# Autodesk Inventor assembly: Fuel Assembly
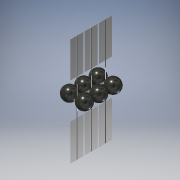
[picture p0: Inventor's stored thumbnail of the model, 180x180]
Saved by Autodesk Inventor 2017.2 (Build 212233000, 233)
## iProperties
Created: 2017-03-31
Part Number: Fuel Assembly
Document SubType Name: Assembly
Designer: haden
Author: haden
## Documents named in this file (5)
- C:\Users\haden\Desktop\Asteroid-Mining-Project\CAD model\Storage Module\Fuel Assembly.iam
- C:\Users\haden\Desktop\Asteroid-Mining-Project\CAD model\Storage Module\Fuel Distributor.ipt
- C:\Users\haden\Desktop\Asteroid-Mining-Project\CAD model\Storage Module\Tube connection.ipt
- C:\Users\haden\Desktop\Asteroid-Mining-Project\CAD model\Storage Module\Tank.ipt
- C:\Users\haden\Desktop\Asteroid-Mining-Project\CAD model\Solar Module\Solar Array.iam
## Components (19 placed, 4 different names)
1. Fuel Distributor:1 — Mate:1, Mate:2, Mate:3, Mate:4, Mate:5, Mate:6, Mate:7, Mate:8, Insert:7, Insert:8, Insert:9, Insert:10, Insert:11, Insert:12
2. Tube connection:1 — Mate:3, Flush:1, Mate:7, Insert:4
3. Tube connection:2 — Mate:2, Flush:1, Flush:2, Insert:5
4. Tube connection:3 — Mate:1, Flush:2, Insert:6
5. Tube connection:4 — Mate:4, Flush:3, Insert:3
6. Tube connection:5 — Mate:5, Flush:3, Flush:4, Insert:2
7. Tube connection:6 — Mate:6, Flush:4, Mate:8, Insert:1
8. Tank:1 — Insert:3
9. Tank:2 — Insert:2
10. Tank:3 — Insert:1
11. Tank:4 — Insert:4
12. Tank:5 — Insert:5
13. Tank:6 — Insert:6
14. Solar Array:1 [sub-assembly] — Insert:7, Angle:1, Angle:2, Angle:3
15. Solar Array:2 [sub-assembly] — Insert:8, Angle:1, Angle:2, Angle:3, Angle:4
16. Solar Array:3 [sub-assembly] — Insert:9, Angle:4, Angle:5
17. Solar Array:4 [sub-assembly] — Insert:12, Angle:5, Angle:6
18. Solar Array:5 [sub-assembly] — Insert:11, Angle:6, Angle:7
19. Solar Array:6 [sub-assembly] — Insert:10, Angle:7
## Relationships (31: Insert 12, Mate 8, Angle 7, Flush 4)
- Mate:1: Fuel Distributor:1 ↔ Tube connection:3
- Mate:2: Fuel Distributor:1 ↔ Tube connection:2
- Mate:3: Fuel Distributor:1 ↔ Tube connection:1
- Mate:4: Fuel Distributor:1 ↔ Tube connection:4
- Mate:5: Fuel Distributor:1 ↔ Tube connection:5
- Mate:6: Fuel Distributor:1 ↔ Tube connection:6
- Flush:1: Tube connection:1 ↔ Tube connection:2
- Flush:2: Tube connection:2 ↔ Tube connection:3
- Flush:3: Tube connection:4 ↔ Tube connection:5
- Flush:4: Tube connection:5 ↔ Tube connection:6
- Mate:7 (-100 mm): Fuel Distributor:1 ↔ Tube connection:1
- Mate:8 (-100 mm): Fuel Distributor:1 ↔ Tube connection:6
- Insert:1: Tube connection:6 ↔ Tank:3
- Insert:2: Tube connection:5 ↔ Tank:2
- Insert:3: Tube connection:4 ↔ Tank:1
- Insert:4: Tube connection:1 ↔ Tank:4
- Insert:5: Tube connection:2 ↔ Tank:5
- Insert:6: Tube connection:3 ↔ Tank:6
- Insert:7: Fuel Distributor:1 ↔ Solar Array:1
- Insert:8: Fuel Distributor:1 ↔ Solar Array:2
- Insert:9: Fuel Distributor:1 ↔ Solar Array:3
- Insert:10: Fuel Distributor:1 ↔ Solar Array:6
- Insert:11: Fuel Distributor:1 ↔ Solar Array:5
- Insert:12: Fuel Distributor:1 ↔ Solar Array:4
- Angle:1 (0 deg): Solar Array:1 ↔ Solar Array:2
- Angle:2 (0 deg): Solar Array:1 ↔ Solar Array:2
- Angle:3 (0 deg): Solar Array:1 ↔ Solar Array:2
- Angle:4 (0 deg): Solar Array:2 ↔ Solar Array:3
- Angle:5 (0 deg): Solar Array:3 ↔ Solar Array:4
- Angle:6 (0 deg): Solar Array:4 ↔ Solar Array:5
- Angle:7 (0 deg): Solar Array:5 ↔ Solar Array:6
